# Autodesk Inventor assembly: Assembly2
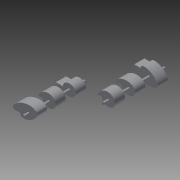
[picture p0: Inventor's stored thumbnail of the model, 180x180]
Saved by Autodesk Inventor 2014 (Build 180170000, 170)
## iProperties
Created: 2014-05-19
Part Number: Assembly2
Document SubType Name: Assembly
Designer: jyesowitz
Author: jyesowitz
## Documents named in this file (5)
- E:\Tech\Final Project first\Assembly2.iam
- E:\Tech\Final Project first\cam 1.ipt
- E:\Tech\Final Project first\cam 2.ipt
- E:\Tech\Final Project first\cam 3.ipt
- E:\Tech\Final Project first\rod.ipt
## Components (8 placed, 4 different names)
1. cam 1:1 — Insert:3
2. cam 2:1 — Insert:1
3. cam 3:1 — Insert:2
4. rod:1 — Insert:1, Insert:2, Insert:3
5. cam 1:2 — Insert:5
6. cam 2:2 — Insert:6
7. cam 3:2 — Insert:4
8. rod:2 — Insert:4, Insert:5, Insert:6
## Relationships (6: Insert 6)
- Insert:1 (25.4 mm): cam 2:1 ↔ rod:1
- Insert:2 (25.4 mm): cam 3:1 ↔ rod:1
- Insert:3 (127 mm): cam 1:1 ↔ rod:1
- Insert:4 (25.4 mm): cam 3:2 ↔ rod:2
- Insert:5 (25.4 mm): cam 1:2 ↔ rod:2
- Insert:6 (127 mm): cam 2:2 ↔ rod:2
